# Autodesk Inventor assembly: chaimber
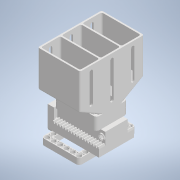
[picture p0: Inventor's stored thumbnail of the model, 180x180]
Saved by Autodesk Inventor 2021 (Build 250183000, 183)
## iProperties
Created: 2024-03-14
Part Number: chaimber
Document SubType Name: Assembly
Designer: 22hamfri
Author: 22hamfri
## Documents named in this file (8)
- C:\Users\22hamfri\Documents\School\Programmering\domino-bil\CAD\chaimber.iam
- C:\Users\22hamfri\Documents\School\Programmering\domino-bil\CAD\chaimber.ipt
- C:\Users\22hamfri\Documents\School\Programmering\domino-bil\CAD\chaimber-adapter.ipt
- C:\Users\22hamfri\Documents\School\Programmering\domino-bil\CAD\magazine-adapter.ipt
- C:\Users\22hamfri\Documents\School\Programmering\domino-bil\CAD\chaimber-bolt.ipt
- C:\Users\22hamfri\Documents\School\Programmering\domino-bil\CAD\bolt-rack.ipt
- C:\Users\22hamfri\Documents\School\Programmering\domino-bil\CAD\magazine-tower.ipt
- C:\Users\22hamfri\Documents\School\Programmering\domino-bil\CAD\vehicle-adapter.ipt
## Components (9 placed, 7 different names)
1. chaimber:1 — Rigid:1, Rigid:2, Angle:1, Mate:1, bolt-action, Rigid:6
2. chaimber-adapter:1 — Rigid:1
3. magazine-adapter:1 — Rigid:2, magazine-attach, Angle:2, Mate:4
4. chaimber-bolt:1 — Angle:1, Mate:1, bolt-action, Rigid:3, Rigid:4
5. bolt-rack:1 — Rigid:3
6. bolt-rack:2 — Rigid:4
7. magazine-tower:1 — Rigid:5
8. magazine-adapter:2 — Rigid:5, magazine-attach, Angle:2, Mate:4
9. vehicle-adapter:1 — Rigid:6
## Relationships (12: WeldJoint 6, Mate 4, Angle 2)
- Rigid:1 [WeldJoint]: chaimber:1 ↔ chaimber-adapter:1
- Rigid:2 [WeldJoint]: chaimber:1 ↔ magazine-adapter:1
- Angle:1 (180 deg): chaimber:1 ↔ chaimber-bolt:1
- Mate:1: chaimber:1 ↔ chaimber-bolt:1
- bolt-action [Mate]: chaimber:1 ↔ chaimber-bolt:1
- Rigid:3 [WeldJoint]: chaimber-bolt:1 ↔ bolt-rack:1
- Rigid:4 [WeldJoint]: chaimber-bolt:1 ↔ bolt-rack:2
- Rigid:5 [WeldJoint]: magazine-tower:1 ↔ magazine-adapter:2
- magazine-attach [Mate]: magazine-adapter:1 ↔ magazine-adapter:2
- Angle:2 (0 deg): magazine-adapter:1 ↔ magazine-adapter:2
- Mate:4: magazine-adapter:1 ↔ magazine-adapter:2
- Rigid:6 [WeldJoint]: chaimber:1 ↔ vehicle-adapter:1
